# Autodesk Inventor assembly: gaming controllbox
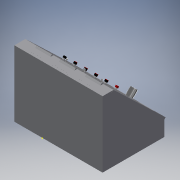
[picture p0: Inventor's stored thumbnail of the model, 180x180]
Saved by Autodesk Inventor 2016 (Build 200138000, 138)
## iProperties
Created: 2016-05-17
Part Number: gaming controllbox
Document SubType Name: Assembly
Designer: Lillahunden
Author: Lillahunden
## Documents named in this file (11)
- C:\Users\Lillahunden\Documents\Inventor\Gaming controllbox\gaming controllbox.iam
- C:\Users\Lillahunden\Documents\Inventor\Gaming controllbox\bottom.ipt
- C:\Users\Lillahunden\Documents\Inventor\Gaming controllbox\back.ipt
- C:\Users\Lillahunden\Documents\Inventor\Gaming controllbox\top.ipt
- C:\Users\Lillahunden\Documents\Inventor\Gaming controllbox\front.ipt
- C:\Users\Lillahunden\Documents\Inventor\Gaming controllbox\left.ipt
- C:\Users\Lillahunden\Documents\Inventor\Gaming controllbox\Frontpanel.ipt
- C:\Users\Lillahunden\Documents\Inventor\Gaming controllbox\ENCODER WHEEL.ipt
- C:\Users\Lillahunden\Documents\Inventor\Gaming controllbox\BLACKBUTTON.ipt
- C:\Users\Lillahunden\Documents\Inventor\Gaming controllbox\REDBUTTON.ipt
- C:\Users\Lillahunden\Documents\Inventor\Gaming controllbox\toggle switch.ipt
## Components (21 placed, 10 different names)
1. bottom:1 — Mate:1, Flush:1, Flush:3, Flush:4, Flush:6
2. back:1 — Mate:1, Flush:1, Flush:2, Flush:7
3. top:1 — Flush:2
4. front:1 — Flush:3, Flush:5
5. left:1 — Flush:4, Flush:8
6. left:2 — Flush:5, Flush:6, Flush:7
7. Frontpanel:1 — Flush:8, Mate:2, Mate:3, Mate:4, Mate:5, Mate:6, Mate:7, Mate:8, Mate:9, Mate:10, Mate:11, Mate:12, Mate:13, Mate:14, Mate:15, Mate:16, Mate:17, Mate:18, Mate:19, Mate:20, Mate:21, Mate:22, Mate:23, Mate:24, Mate:25, Mate:26, Mate:27, Mate:28, Mate:29
8. ENCODER WHEEL:1 — Mate:28, Mate:29
9. BLACKBUTTON:1 — Mate:5, Mate:9
10. BLACKBUTTON:2 — Mate:6, Mate:10
11. BLACKBUTTON:3 — Mate:4, Mate:8
12. BLACKBUTTON:4 — Mate:7, Mate:11
13. BLACKBUTTON:5 — Mate:2, Mate:3
14. REDBUTTON:1 — Mate:13, Mate:22
15. REDBUTTON:2 — Mate:14, Mate:24
16. REDBUTTON:3 — Mate:15, Mate:20
17. REDBUTTON:4 — Mate:16, Mate:21
18. REDBUTTON:5 — Mate:12, Mate:23
19. toggle switch:1 — Mate:17, Mate:26
20. toggle switch:2 — Mate:19, Mate:25
21. toggle switch:3 — Mate:18, Mate:27
## Relationships (37: Mate 29, Flush 8)
- Mate:1: bottom:1 ↔ back:1
- Flush:1: bottom:1 ↔ back:1
- Flush:2: back:1 ↔ top:1
- Flush:3: bottom:1 ↔ front:1
- Flush:4: bottom:1 ↔ left:1
- Flush:5: front:1 ↔ left:2
- Flush:6: bottom:1 ↔ left:2
- Flush:7: back:1 ↔ left:2
- Flush:8: left:1 ↔ Frontpanel:1
- Mate:2: Frontpanel:1 ↔ BLACKBUTTON:5
- Mate:3: Frontpanel:1 ↔ BLACKBUTTON:5
- Mate:4: Frontpanel:1 ↔ BLACKBUTTON:3
- Mate:5: Frontpanel:1 ↔ BLACKBUTTON:1
- Mate:6: Frontpanel:1 ↔ BLACKBUTTON:2
- Mate:7: Frontpanel:1 ↔ BLACKBUTTON:4
- Mate:8: Frontpanel:1 ↔ BLACKBUTTON:3
- Mate:9: Frontpanel:1 ↔ BLACKBUTTON:1
- Mate:10: Frontpanel:1 ↔ BLACKBUTTON:2
- Mate:11: Frontpanel:1 ↔ BLACKBUTTON:4
- Mate:12: Frontpanel:1 ↔ REDBUTTON:5
- Mate:13: Frontpanel:1 ↔ REDBUTTON:1
- Mate:14: Frontpanel:1 ↔ REDBUTTON:2
- Mate:15: Frontpanel:1 ↔ REDBUTTON:3
- Mate:16: Frontpanel:1 ↔ REDBUTTON:4
- Mate:17: Frontpanel:1 ↔ toggle switch:1
- Mate:18: Frontpanel:1 ↔ toggle switch:3
- Mate:19: Frontpanel:1 ↔ toggle switch:2
- Mate:20: Frontpanel:1 ↔ REDBUTTON:3
- Mate:21: Frontpanel:1 ↔ REDBUTTON:4
- Mate:22: Frontpanel:1 ↔ REDBUTTON:1
- Mate:23: Frontpanel:1 ↔ REDBUTTON:5
- Mate:24: Frontpanel:1 ↔ REDBUTTON:2
- Mate:25: Frontpanel:1 ↔ toggle switch:2
- Mate:26: Frontpanel:1 ↔ toggle switch:1
- Mate:27: Frontpanel:1 ↔ toggle switch:3
- Mate:28 (1 mm): Frontpanel:1 ↔ ENCODER WHEEL:1
- Mate:29: Frontpanel:1 ↔ ENCODER WHEEL:1
